# Autodesk Inventor assembly: Robot
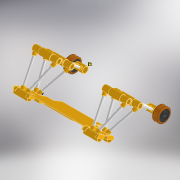
[picture p0: Inventor's stored thumbnail of the model, 180x180]
Saved by Autodesk Inventor 2021 (Build 250183000, 183)
## iProperties
Created: 2024-02-19
Part Number: Robot
Document SubType Name: Assembly
Designer: Martin
Author: Martin
## Documents named in this file (18)
- C:\Users\ASUS\OneDrive - Universidad de Antioquia\2024-1\Robótica\CAD\Robot2.iam
- C:\Users\ASUS\OneDrive - Universidad de Antioquia\2024-1\Robótica\CAD\JuntaRodilla.ipt
- C:\Users\ASUS\OneDrive - Universidad de Antioquia\2024-1\Robótica\CAD\SoporteMotor.ipt
- C:\Users\ASUS\OneDrive - Universidad de Antioquia\2024-1\Robótica\CAD\Tubo1.ipt
- C:\Users\ASUS\OneDrive - Universidad de Antioquia\2024-1\Robótica\CAD\Tubo2.ipt
- C:\Users\ASUS\OneDrive - Universidad de Antioquia\2024-1\Robótica\CAD\EjeRodilla.ipt
- C:\Users\ASUS\OneDrive - Universidad de Antioquia\2024-1\Robótica\CAD\JuntaEjeCadera.ipt
- C:\Users\ASUS\OneDrive - Universidad de Antioquia\2024-1\Robótica\CAD\Tubo3.ipt
- C:\Users\ASUS\OneDrive - Universidad de Antioquia\2024-1\Robótica\CAD\Tubo4.ipt
- C:\Users\ASUS\OneDrive - Universidad de Antioquia\2024-1\Robótica\CAD\JuntaRodilla2.ipt
- C:\Users\ASUS\OneDrive - Universidad de Antioquia\2024-1\Robótica\CAD\JuntaEje2Trasero.ipt
- C:\Users\ASUS\OneDrive - Universidad de Antioquia\2024-1\Robótica\CAD\EjeRodilla2.ipt
- C:\Users\ASUS\OneDrive - Universidad de Antioquia\2024-1\Robótica\CAD\Tubo5.ipt
- C:\Users\ASUS\OneDrive - Universidad de Antioquia\2024-1\Robótica\CAD\Tubo6.ipt
- C:\Users\ASUS\OneDrive - Universidad de Antioquia\2024-1\Robótica\CAD\JuntaCadera.ipt
- C:\Users\ASUS\OneDrive - Universidad de Antioquia\2024-1\Robótica\CAD\JuntaTrasero.ipt
- C:\Users\ASUS\OneDrive - Universidad de Antioquia\2024-1\Robótica\CAD\ChasisCircuiteria.ipt
- C:\Users\ASUS\OneDrive - Universidad de Antioquia\2024-1\Robótica\CAD\Llanta.ipt
## Components (41 placed, 17 different names)
1. JuntaRodilla:1 — Mate:5, Mate:6, Mate:7, Mate:11, Mate:12, Mate:13, Mate:14, Mate:23
2. SoporteMotor:1 — Mate:1, Mate:2, Mate:3, Mate:4, Mate:87, Angle:1, Angle:3, Mate:88
3. Tubo1:1 — Mate:1, Mate:2, Mate:5
4. Tubo2:1 — Mate:3, Mate:4, Mate:6, Angle:3, Angle:4
5. EjeRodilla:1 — Mate:7, Mate:9, Mate:10, Mate:21, Mate:22, Angle:2
6. JuntaEjeCadera:1 — Mate:9, Mate:10, Mate:32, Mate:35, Angle:2, Angle:4
7. Tubo3:1 — Mate:11, Mate:12, Mate:15
8. Tubo4:1 — Mate:13, Mate:14, Mate:16
9. JuntaRodilla2:1 — Mate:15, Mate:16, Mate:27, Mate:30
10. JuntaEje2Trasero:1 — Mate:25, Mate:26, Mate:34, Mate:38
11. JuntaEjeCadera:2 — Mate:21, Mate:22, Mate:23, Mate:31, Mate:36
12. EjeRodilla2:1 — Mate:25, Mate:26, Mate:27, Mate:28, Mate:29
13. JuntaEje2Trasero:2 — Mate:28, Mate:29, Mate:30, Mate:33, Mate:37
14. Tubo5:1 — Mate:31, Mate:36, Mate:39
15. Tubo6:1 — Mate:34, Mate:38, Mate:41
16. Tubo5:2 — Mate:32, Mate:35, Mate:40
17. Tubo6:2 — Mate:33, Mate:37, Mate:42
18. JuntaCadera:1 — Mate:39, Mate:40, Mate:45, Mate:46
19. JuntaTrasero:1 — Mate:41, Mate:42, Mate:43
20. ChasisCircuiteria:1 — Mate:43, Mate:45, Mate:46, Mate:125, Mate:126, Mate:127
21. Llanta:2 — Mate:87, Mate:88
22. JuntaRodilla:2
23. SoporteMotor:2 — Mate:128, Mate:129
24. Tubo1:2
25. Tubo2:2
26. EjeRodilla:2
27. JuntaEjeCadera:3
28. Tubo3:2
29. Tubo4:2
30. JuntaRodilla2:2
31. JuntaEje2Trasero:3
32. JuntaEjeCadera:4
33. EjeRodilla2:2
34. JuntaEje2Trasero:4
35. Tubo5:3
36. Tubo6:3
37. Tubo5:4
38. Tubo6:4
39. JuntaCadera:2 — Mate:125, Mate:126
40. JuntaTrasero:2 — Mate:127
41. Llanta:3 — Mate:128, Mate:129
## Relationships (89: Mate 82, Angle 7)
- Mate:1: SoporteMotor:1 ↔ Tubo1:1
- Mate:2 (-20 mm): SoporteMotor:1 ↔ Tubo1:1
- Mate:3: SoporteMotor:1 ↔ Tubo2:1
- Mate:4 (-20 mm): SoporteMotor:1 ↔ Tubo2:1
- Mate:5: JuntaRodilla:1 ↔ Tubo1:1
- Mate:6: JuntaRodilla:1 ↔ Tubo2:1
- Mate:7: JuntaRodilla:1 ↔ EjeRodilla:1
- Mate:9: EjeRodilla:1 ↔ JuntaEjeCadera:1
- Mate:10: EjeRodilla:1 ↔ JuntaEjeCadera:1
- Mate:11: JuntaRodilla:1 ↔ Tubo3:1
- Mate:12 (-15 mm): JuntaRodilla:1 ↔ Tubo3:1
- Mate:13: JuntaRodilla:1 ↔ Tubo4:1
- Mate:14 (-15 mm): JuntaRodilla:1 ↔ Tubo4:1
- Mate:15: Tubo3:1 ↔ JuntaRodilla2:1
- Mate:16: Tubo4:1 ↔ JuntaRodilla2:1
- Mate:21: EjeRodilla:1 ↔ JuntaEjeCadera:2
- Mate:22: EjeRodilla:1 ↔ JuntaEjeCadera:2
- Mate:23: JuntaRodilla:1 ↔ JuntaEjeCadera:2
- Mate:25: JuntaEje2Trasero:1 ↔ EjeRodilla2:1
- Mate:26: JuntaEje2Trasero:1 ↔ EjeRodilla2:1
- Mate:27: JuntaRodilla2:1 ↔ EjeRodilla2:1
- Mate:28: EjeRodilla2:1 ↔ JuntaEje2Trasero:2
- Mate:29: EjeRodilla2:1 ↔ JuntaEje2Trasero:2
- Mate:30: JuntaRodilla2:1 ↔ JuntaEje2Trasero:2
- Mate:31: JuntaEjeCadera:2 ↔ Tubo5:1
- Mate:32: JuntaEjeCadera:1 ↔ Tubo5:2
- Mate:33: JuntaEje2Trasero:2 ↔ Tubo6:2
- Mate:34: JuntaEje2Trasero:1 ↔ Tubo6:1
- Mate:35 (-15 mm): JuntaEjeCadera:1 ↔ Tubo5:2
- Mate:36 (-15 mm): JuntaEjeCadera:2 ↔ Tubo5:1
- Mate:37 (-15 mm): JuntaEje2Trasero:2 ↔ Tubo6:2
- Mate:38 (-15 mm): JuntaEje2Trasero:1 ↔ Tubo6:1
- Mate:39: Tubo5:1 ↔ JuntaCadera:1
- Mate:40: Tubo5:2 ↔ JuntaCadera:1
- Mate:41: Tubo6:1 ↔ JuntaTrasero:1
- Mate:42: Tubo6:2 ↔ JuntaTrasero:1
- Mate:43: JuntaTrasero:1 ↔ ChasisCircuiteria:1
- Mate:45: JuntaCadera:1 ↔ ChasisCircuiteria:1
- Mate:46 (1 mm): JuntaCadera:1 ↔ ChasisCircuiteria:1
- Mate:87: SoporteMotor:1 ↔ Llanta:2
- Angle:1 (-50 deg): SoporteMotor:1
- Angle:2 (0 deg): EjeRodilla:1 ↔ JuntaEjeCadera:1
- Angle:3 (0 deg): SoporteMotor:1 ↔ Tubo2:1
- Angle:4 (100 deg): Tubo2:1 ↔ JuntaEjeCadera:1
- Mate:88: SoporteMotor:1 ↔ Llanta:2
- [Mate]: SoporteMotor:2 ↔ Tubo1:2
- [Mate] (-20 mm): SoporteMotor:2 ↔ Tubo1:2
- [Mate]: SoporteMotor:2 ↔ Tubo2:2
- [Mate] (-20 mm): SoporteMotor:2 ↔ Tubo2:2
- [Mate]: JuntaRodilla:2 ↔ Tubo1:2
- [Mate]: JuntaRodilla:2 ↔ Tubo2:2
- [Mate]: JuntaRodilla:2 ↔ EjeRodilla:2
- [Mate]: EjeRodilla:2 ↔ JuntaEjeCadera:3
- [Mate]: EjeRodilla:2 ↔ JuntaEjeCadera:3
- [Mate]: JuntaRodilla:2 ↔ Tubo3:2
- [Mate] (-15 mm): JuntaRodilla:2 ↔ Tubo3:2
- [Mate]: JuntaRodilla:2 ↔ Tubo4:2
- [Mate] (-15 mm): JuntaRodilla:2 ↔ Tubo4:2
- [Mate]: Tubo3:2 ↔ JuntaRodilla2:2
- [Mate]: Tubo4:2 ↔ JuntaRodilla2:2
- [Mate]: EjeRodilla:2 ↔ JuntaEjeCadera:4
- [Mate]: EjeRodilla:2 ↔ JuntaEjeCadera:4
- [Mate]: JuntaRodilla:2 ↔ JuntaEjeCadera:4
- [Mate]: JuntaEje2Trasero:3 ↔ EjeRodilla2:2
- [Mate]: JuntaEje2Trasero:3 ↔ EjeRodilla2:2
- [Mate]: JuntaRodilla2:2 ↔ EjeRodilla2:2
- [Mate]: EjeRodilla2:2 ↔ JuntaEje2Trasero:4
- [Mate]: EjeRodilla2:2 ↔ JuntaEje2Trasero:4
- [Mate]: JuntaRodilla2:2 ↔ JuntaEje2Trasero:4
- [Mate]: JuntaEjeCadera:4 ↔ Tubo5:3
- [Mate]: JuntaEjeCadera:3 ↔ Tubo5:4
- [Mate]: JuntaEje2Trasero:4 ↔ Tubo6:4
- [Mate]: JuntaEje2Trasero:3 ↔ Tubo6:3
- [Mate] (-15 mm): JuntaEjeCadera:3 ↔ Tubo5:4
- [Mate] (-15 mm): JuntaEjeCadera:4 ↔ Tubo5:3
- [Mate] (-15 mm): JuntaEje2Trasero:4 ↔ Tubo6:4
- [Mate] (-15 mm): JuntaEje2Trasero:3 ↔ Tubo6:3
- [Mate]: Tubo5:3 ↔ JuntaCadera:2
- [Mate]: Tubo5:4 ↔ JuntaCadera:2
- [Mate]: Tubo6:3 ↔ JuntaTrasero:2
- [Mate]: Tubo6:4 ↔ JuntaTrasero:2
- [Angle] (0 deg): EjeRodilla:2 ↔ JuntaEjeCadera:3
- [Angle] (0 deg): SoporteMotor:2 ↔ Tubo2:2
- [Angle] (100 deg): Tubo2:2 ↔ JuntaEjeCadera:3
- Mate:125: ChasisCircuiteria:1 ↔ JuntaCadera:2
- Mate:126 (1 mm): ChasisCircuiteria:1 ↔ JuntaCadera:2
- Mate:127: ChasisCircuiteria:1 ↔ JuntaTrasero:2
- Mate:128: SoporteMotor:2 ↔ Llanta:3
- Mate:129: SoporteMotor:2 ↔ Llanta:3
## Named parameters: d117_d114 = 0 deg, d118_d115 = 100 deg, d119_d0 = 0 mm, d120_d1 = -20 mm, d121_d2 = 0 mm, d122_d3 = -20 mm, d123_d4 = 0 mm, d124_d112 = 0 deg, d125_d50 = 0 mm, d126_d51 = 0 mm, d127_d52 = 0 mm, d128_d53 = 0 mm, d129_d54 = -15 mm, d130_d55 = -15 mm, d131_d56 = -15 mm, d132_d57 = -15 mm, d133_d58 = 0 mm, d134_d59 = 0 mm, d135_d60 = 0 mm, d136_d61 = 0 mm, d137_d5 = 0 mm, d138_d6 = 0 mm, d139_d17 = 0 mm, d140_d18 = 0 mm, d141_d25 = 0 mm, d142_d26 = -15 mm, d143_d27 = 0 mm, d144_d28 = -15 mm, d145_d31 = 0 mm, d146_d32 = 0 mm, d147_d39 = 0 mm, d148_d40 = 0 mm, d149_d41 = 0 mm, d150_d44 = 0 mm, d151_d45 = 0 mm, d152_d46 = 0 mm, d153_d47 = 0 mm, d154_d48 = 0 mm, d155_d49 = 0 mm
